# Autodesk Inventor assembly: dlc
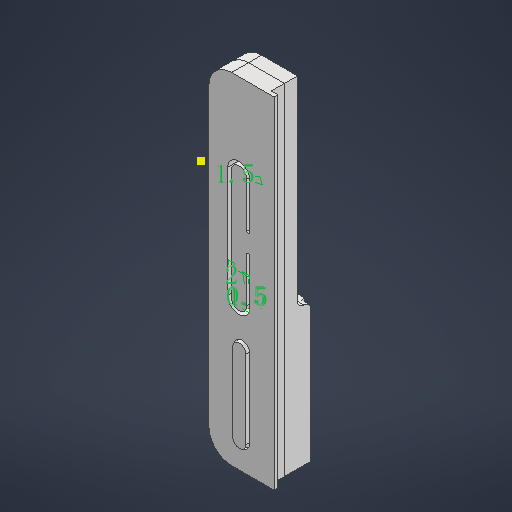
[picture p0: Inventor's stored thumbnail of the model, 512x512]
Saved by Autodesk Inventor 2025 (Build 290162000, 162)
## iProperties
Created: 2025-11-18
Part Number: dlc
Document SubType Name: Assembly
Designer: XH
Author: XH
## Documents named in this file (5)
- D:\三星\dlc.iam
- D:\三星\电子\音量接口.ipt
- D:\三星\电子\指纹识别.ipt
- D:\三星\指纹dlc.ipt
- D:\三星\指纹安装板.ipt
## Components (4 placed, 4 different names)
1. 音量接口:1 — 表面齐平:1
2. 指纹识别:1 — 配合:1
3. 指纹dlc:1 — 配合:1, 表面齐平:1, 表面齐平:2, 表面齐平:3, 配合:2, 配合:3
4. 指纹安装板:1 — 表面齐平:2, 表面齐平:3, 配合:2, 配合:3
## Relationships (6: Mate 3, Flush 3)
- 配合:1 [Mate]: 指纹识别:1 ↔ 指纹dlc:1
- 表面齐平:1 [Flush]: 音量接口:1 ↔ 指纹dlc:1
- 表面齐平:2 [Flush]: 指纹dlc:1 ↔ 指纹安装板:1
- 表面齐平:3 [Flush]: 指纹dlc:1 ↔ 指纹安装板:1
- 配合:2 [Mate]: 指纹dlc:1 ↔ 指纹安装板:1
- 配合:3 [Mate]: 指纹dlc:1 ↔ 指纹安装板:1
